# Autodesk Inventor assembly: Assembly2
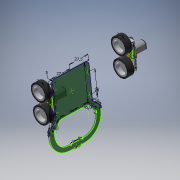
[picture p0: Inventor's stored thumbnail of the model, 180x180]
Saved by Autodesk Inventor 2016 (Build 200138000, 138)
## iProperties
Created: 2017-05-26
Part Number: Assembly2
Material: Ogólny
Document SubType Name: Assembly
Designer: Karol
Author: Karol
## Documents named in this file (8)
- D:\ele\MicroMouse\v2\Assembly2.iam
- D:\ele\MicroMouse\v2\wheel.ipt
- D:\ele\MicroMouse\v2\togh.ipt
- D:\ele\MicroMouse\v2\bolt.ipt
- D:\ele\MicroMouse\v2\tyre.ipt
- D:\ele\MicroMouse\v2\motor.ipt
- D:\ele\MicroMouse\v2\magnet.ipt
- D:\ele\MicroMouse\v2\mainpcb.ipt
## Components (21 placed, 7 different names)
1. mainpcb:1 — Mate:1
2. bolt:3
3. bolt:4
4. wheel:3
5. wheel:4
6. magnet:3
7. magnet:4
8. togh:2 — Mate:1
9. tyre:3
10. tyre:4
11. motor:2
12. bolt:5
13. bolt:6
14. wheel:5
15. wheel:6
16. magnet:5
17. magnet:6
18. togh:3
19. tyre:5
20. tyre:6
21. motor:3
## Relationships (19: WeldJoint 18, Mate 1)
- [WeldJoint]: bolt:4 ↔ wheel:4
- [WeldJoint]: bolt:3 ↔ wheel:3
- [WeldJoint]: bolt:3 ↔ magnet:3
- [WeldJoint]: bolt:4 ↔ magnet:4
- [WeldJoint]: bolt:4 ↔ togh:2
- [WeldJoint] (-5 mm): bolt:3 ↔ togh:2
- [WeldJoint]: wheel:3 ↔ tyre:3
- [WeldJoint]: wheel:4 ↔ tyre:4
- [WeldJoint]: togh:2 ↔ motor:2
- Mate:1: mainpcb:1 ↔ togh:2
- [WeldJoint]: bolt:6 ↔ wheel:6
- [WeldJoint]: bolt:5 ↔ wheel:5
- [WeldJoint]: bolt:5 ↔ magnet:5
- [WeldJoint]: bolt:6 ↔ magnet:6
- [WeldJoint]: bolt:6 ↔ togh:3
- [WeldJoint] (-5 mm): bolt:5 ↔ togh:3
- [WeldJoint]: wheel:5 ↔ tyre:5
- [WeldJoint]: wheel:6 ↔ tyre:6
- [WeldJoint]: togh:3 ↔ motor:3
## Named parameters: d102_d99 = 0 mm, d103_d100 = -5 mm, d104_d101 = 0 mm, d105_d68 = 0 mm, d106_d67 = 0 mm, d107_d21 = 7.108573 deg, d108_d22 = -0.02503 mm, d109_d23 = 0.199983 deg, d110_d24 = -4.88726 mm, d111_d4 = 0 mm, d112_d5 = 0.127925 deg, d113_d6 = 0 mm, d114_d7 = -6.839272 deg, d115_d12 = 0 mm, d116_d13 = 6.940569 deg, d117_d14 = 0 mm, d118_d15 = 2.56641 deg, d129_d102_d99 = 0 mm, d130_d103_d100 = -5 mm, d131_d104_d101 = 0 mm, d132_d105_d68 = 0 mm, d133_d106_d67 = 0 mm, d134_d107_d21 = 7.108573 deg, d135_d108_d22 = -0.02503 mm, d136_d109_d23 = 0.199983 deg, d137_d110_d24 = -4.88726 mm, d138_d111_d4 = 0 mm, d139_d112_d5 = 0.127925 deg, d140_d113_d6 = 0 mm, d141_d114_d7 = -6.839272 deg, d142_d115_d12 = 0 mm, d143_d116_d13 = 6.940569 deg, d144_d117_d14 = 0 mm, d145_d118_d15 = 2.56641 deg
